# Autodesk Inventor assembly: 3dPrinter
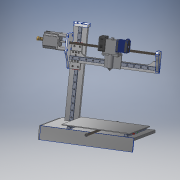
[picture p0: Inventor's stored thumbnail of the model, 180x180]
Saved by Autodesk Inventor 2019 (Build 230136000, 136)
## iProperties
Created: 2018-10-03
Part Number: 3dPrinter
Document SubType Name: Assembly
Designer: LillaHunden
Mass: 6608.48 g
Surface Area: 8581.85 cm^2
Volume: 2705.8 cm^3
Density: 2.44234 g/cm^3
Author: LillaHunden
## Documents named in this file (40)
- C:\Users\LillaHunden\Documents\Inventor\3dprinter\3dPrinter\3dPrinter.iam
- C:\Users\LillaHunden\Documents\Inventor\3dprinter\3dPrinter\baseplate.ipt
- C:\Users\LillaHunden\Documents\Inventor\3dprinter\3dPrinter\Zcolumn.ipt
- C:\Users\LillaHunden\Documents\Inventor\3dprinter\3dPrinter\ZcolStiffer.ipt
- C:\Users\LillaHunden\Documents\Inventor\3dprinter\3dPrinter\Linear Rials import\Rail Z.ipt
- C:\Users\LillaHunden\Documents\Inventor\3dprinter\3dPrinter\Linear Rials import\hotplate.ipt
- C:\Users\LillaHunden\Documents\Inventor\3dprinter\3dPrinter\Linear Rials import\MGN block.iam
- C:\Users\LillaHunden\Documents\Inventor\3dprinter\3dPrinter\Linear Rials import\Rail Y.ipt
- C:\Users\LillaHunden\Documents\Inventor\3dprinter\3dPrinter\Linear Rials import\Xcolum.ipt
- C:\Users\LillaHunden\Documents\Inventor\3dprinter\3dPrinter\Linear Rials import\XcolBracket.ipt
- C:\Users\LillaHunden\Documents\Inventor\3dprinter\3dPrinter\Linear Rials import\Rail X.ipt
- C:\Users\LillaHunden\Documents\Inventor\3dprinter\3dPrinter\Design Accelerator\Bolted Connection2.iam
- C:\Users\LillaHunden\Documents\Inventor\3dprinter\3dPrinter\Linear Rials import\Trapezoidal lead screw tr8x8-4 X.ipt
- C:\Users\LillaHunden\Documents\Inventor\3dprinter\3dPrinter\Linear Rials import\Trapezoidal lead screw tr8x8-4 Y.ipt
- C:\Users\LillaHunden\Documents\Inventor\3dprinter\3dPrinter\Linear Rials import\Trapezoidal lead screw tr8x8-4 Z.ipt
- C:\Users\LillaHunden\Documents\Inventor\3dprinter\3dPrinter\Linear Rials import\TR8_8(P4) Antibacklash Nut w. spring.ipt
- C:\Users\LillaHunden\Documents\Inventor\3dprinter\3dPrinter\Linear Rials import\ZnutBracket.ipt
- C:\Users\LillaHunden\Documents\Inventor\3dprinter\3dPrinter\Design Accelerator\Bolted Connection3.iam
- C:\Users\LillaHunden\Documents\Inventor\3dprinter\3dPrinter\Design Accelerator\Bolted Connection4.iam
- C:\Users\LillaHunden\Documents\Inventor\3dprinter\3dPrinter\ZBaringBracket.ipt
- C:\Users\LillaHunden\Documents\Inventor\3dprinter\3dPrinter\XMotorMount.ipt
- C:\Users\LillaHunden\Documents\Inventor\3dprinter\3dPrinter\23hs6403.ipt
- C:\Users\LillaHunden\Documents\Inventor\3dprinter\3dPrinter\Pulley import\GT2-20T-9mm\GT2_20T_9mm.ipt
- C:\Users\LillaHunden\Documents\Inventor\3dprinter\3dPrinter\XbearingBracket.ipt
- C:\Users\LillaHunden\Documents\Inventor\3dprinter\3dPrinter\3dPrinter\Design Accelerator\Bolted Connection1.iam
- C:\Users\LillaHunden\Documents\Inventor\3dprinter\3dPrinter\3dPrinter\Design Accelerator\Bolted Connection2.iam
- C:\Users\LillaHunden\Documents\Inventor\3dprinter\3dPrinter\3dPrinter\Design Accelerator\Bolted Connection3.iam
- C:\Users\LillaHunden\Documents\Inventor\3dprinter\3dPrinter\MR115 2RS.ipt
- C:\Users\LillaHunden\Documents\Inventor\3dprinter\3dPrinter\Extruder.iam
- C:\Users\LillaHunden\Documents\Inventor\3dprinter\3dPrinter\Extruder bracket.ipt
- C:\Users\LillaHunden\Documents\Inventor\Content Center Files\R2019\en-US\DIN 912\DIN 912 - M3 x 0,5 x 5 x 3,75.ipt
- C:\Users\LillaHunden\Documents\Inventor\3dprinter\3dPrinter\Frame Bottom Front.ipt
- C:\Users\LillaHunden\Documents\Inventor\3dprinter\3dPrinter\Frame bottom Left.ipt
- C:\Users\LillaHunden\Documents\Inventor\3dprinter\3dPrinter\3dPrinter\Design Accelerator\Bolted Connection4.iam
- C:\Users\LillaHunden\Documents\Inventor\3dprinter\3dPrinter\XMotorStandoff.ipt
- C:\Users\LillaHunden\Documents\Inventor\3dprinter\3dPrinter\3dPrinter\Design Accelerator\Bolted Connection6.iam
- C:\Users\LillaHunden\Documents\Inventor\3dprinter\3dPrinter\3dPrinter\Design Accelerator\Bolted Connection9.iam
- C:\Users\LillaHunden\Documents\Inventor\3dprinter\3dPrinter\3dPrinter\Design Accelerator\Bolted Connection10.iam
- C:\Users\LillaHunden\Documents\Inventor\3dprinter\3dPrinter\3dPrinter\Design Accelerator\Bolted Connection8.iam
- C:\Users\LillaHunden\Documents\Inventor\3dprinter\3dPrinter\XGuideBracket.ipt
## Components (63 placed, 29 different names)
1. baseplate:1 — Mate:20, Angle:1, Angle:2, Angle:3, Mate:32, Flush:16, Flush:17, Flush:25, Flush:26, Angle:11, Angle:12, Flush:40, Flush:41
2. Zcolumn:1 — Mate:11, Mate:12, Flush:8, Mate:20, Mate:21, Flush:9, Mate:22, Angle:3, Angle:4, Flush:25, Flush:26, Angle:7, Flush:30, Flush:31
3. ZcolStiffer:1 — Mate:11, Mate:12, Flush:8
4. Rail Z:1 — Mate:21, Flush:9, Mate:22, Mate:25, Mate:26, Mate:85, Mate:86
5. hotplate:1 — Mate:23, Mate:24, Flush:10, Flush:12, Angle:1, Angle:2, Flush:17, Angle:15
6. MGN block:1 [sub-assembly] — Mate:25, Angle:4, Mate:26, Flush:13, Mate:27, Flush:14, Flush:18, Flush:19, Flush:22, Mate:115, Mate:117
7. MGN block:2 [sub-assembly] — Flush:13, Mate:27, Flush:14
8. MGN block:3 [sub-assembly] — Mate:23, Flush:11, Symmetry:1, Flush:12, Mate:28, Mate:29
9. MGN block:4 [sub-assembly] — Mate:24, Flush:10, Flush:11, Symmetry:1, Mate:30, Mate:31
10. Rail Y:1 — Mate:30, Mate:31, Flush:15
11. Rail Y:2 — Mate:28, Mate:29, Flush:15, Mate:32, Flush:16, Angle:6
12. Xcolum:1 — Mate:33, Flush:20, Flush:21, Mate:34, Flush:23, Flush:24, Angle:5, Flush:29, Flush:36, Flush:37, Mate:116, Mate:118, Mate:119, Flush:44, Flush:45, Flush:49
13. XcolBracket:1 — Flush:18, Flush:19, Mate:33, Flush:20, Flush:21, Flush:22, Mate:50, Flush:33, Flush:34, Mate:114
14. Rail X:1 — Mate:34, Flush:23, Flush:24, Mate:35, Mate:36, Mate:102, Mate:103
15. MGN block:5 [sub-assembly] — Mate:35, Mate:36, Angle:16, Flush:39, Mate:76, Mate:77, Mate:125
16. Bolted Connection:1 [sub-assembly] — Mate:114, Mate:115
17. Trapezoidal lead screw tr8x8-4 X:1 — Angle:5, Mate:40, Mate:79, Mate:80
18. Trapezoidal lead screw tr8x8-4 Y:1 — Angle:6, Mate:41, Mate:58, Mate:73, Mate:74
19. Trapezoidal lead screw tr8x8-4 Z:1 — Angle:7, Mate:39, Mate:56, Mate:71
20. TR8_8(P4) Antibacklash Nut w. spring:1 — Mate:39, Mate:47, Mate:84
21. TR8_8(P4) Antibacklash Nut w. spring:2 — Mate:40
22. TR8_8(P4) Antibacklash Nut w. spring:3 — Mate:41
23. ZnutBracket:1 — Flush:29, Mate:47, Mate:83, Mate:104, Mate:105
24. Bolted Connection:2 [sub-assembly] — Mate:104, Mate:105
25. Bolted Connection:3 [sub-assembly] — Mate:83, Mate:84
26. ZBaringBracket:1 — Flush:30, Flush:31, Mate:61, Mate:62, Mate:63, Mate:64, Mate:69, Mate:70
27. XMotorMount:1 — Mate:50, Flush:33, Flush:34, Mate:78, Flush:42, Angle:17, Flush:43, Mate:120, Mate:121, Insert:9
28. 23hs6403:1 — Mate:78, Mate:79, Mate:80, Mate:93, Mate:94, Mate:95, Mate:96, Mate:97, Mate:98, Angle:17, Flush:43
29. 23hs6403:2 — Angle:12, Angle:13, Mate:57
30. 23hs6403:3 — Mate:56, Angle:11
31. GT2_20T_9mm:3 — Angle:14, Mate:58
32. GT2_20T_9mm:4 — Angle:13, Mate:57, Angle:14
33. XbearingBracket:1 — Flush:36, Flush:37, Flush:44, Flush:45, Mate:122, Mate:123, Mate:124
34. Bolted Connection:4 [sub-assembly] — Mate:61, Mate:62
35. Bolted Connection:5 [sub-assembly] — Mate:63, Mate:64
36. Bolted Connection:6 [sub-assembly] — Mate:85, Mate:86
37. MR115 2RS:1 — Mate:73
38. MR115 2RS:2 — Mate:122
39. MR115 2RS:3 — Mate:69, Mate:70, Mate:71
40. MR115 2RS:4 — Mate:74
41. Extruder:1 [sub-assembly] — Angle:15, Angle:16, Flush:38
42. Extruder bracket:1 — Flush:38, Insert:1, Insert:2, Insert:3, Insert:4, Insert:5, Insert:6, Insert:7, Insert:8, Flush:39, Mate:76, Mate:77, Flush:46, Flush:47, Flush:48
43. DIN 912 - replaced by DIN EN ISO 4762 M3 x 5:1 — Insert:1
44. DIN 912 - replaced by DIN EN ISO 4762 M3 x 5:2 — Insert:2
45. DIN 912 - replaced by DIN EN ISO 4762 M3 x 5:3 — Insert:3
46. DIN 912 - replaced by DIN EN ISO 4762 M3 x 5:4 — Insert:4
47. DIN 912 - replaced by DIN EN ISO 4762 M3 x 5:5 — Insert:5
48. DIN 912 - replaced by DIN EN ISO 4762 M3 x 5:6 — Insert:6
49. DIN 912 - replaced by DIN EN ISO 4762 M3 x 5:7 — Insert:7
50. DIN 912 - replaced by DIN EN ISO 4762 M3 x 5:8 — Insert:8
51. Frame Bottom Front:1 — Flush:40
52. Frame bottom Left:1 — Flush:41
53. Bolted Connection:7 [sub-assembly] — Mate:102, Mate:103
54. XMotorStandoff:1 — Flush:42
55. XMotorStandoff:2 — Mate:96, Mate:97
56. XMotorStandoff:3 — Mate:95, Mate:98
57. XMotorStandoff:4 — Mate:93, Mate:94
58. Bolted Connection:8 [sub-assembly] — Mate:120, Mate:121
59. Bolted Connection:10 [sub-assembly] — Mate:116, Mate:117
60. Bolted Connection:11 [sub-assembly] — Mate:118, Mate:119
61. MR115 2RS:5 — Insert:9
62. Bolted Connection:12 [sub-assembly] — Mate:123, Mate:124
63. XGuideBracket:1 — Mate:125, Flush:46, Flush:47, Flush:48, Flush:49
## Relationships (129: Mate 67, Flush 38, Angle 14, Insert 9, Symmetry 1)
- Mate:11: Zcolumn:1 ↔ ZcolStiffer:1
- Mate:12: Zcolumn:1 ↔ ZcolStiffer:1
- Flush:8: Zcolumn:1 ↔ ZcolStiffer:1
- Mate:20 (-5 mm): baseplate:1 ↔ Zcolumn:1
- Mate:21: Zcolumn:1 ↔ Rail Z:1
- Flush:9 (7 mm): Zcolumn:1 ↔ Rail Z:1
- Mate:22: Zcolumn:1 ↔ Rail Z:1
- Mate:23: hotplate:1 ↔ MGN block:3
- Mate:24: hotplate:1 ↔ MGN block:4
- Flush:10 (83 mm): hotplate:1 ↔ MGN block:4
- Flush:11: MGN block:3 ↔ MGN block:4
- Symmetry:1: MGN block:3 ↔ MGN block:4
- Flush:12 (7 mm): hotplate:1 ↔ MGN block:3
- Angle:1 (180 deg): baseplate:1 ↔ hotplate:1
- Angle:2 (90 deg): baseplate:1 ↔ hotplate:1
- Angle:3 (0 deg): baseplate:1 ↔ Zcolumn:1
- Mate:25: Rail Z:1 ↔ MGN block:1
- Angle:4 (0 deg): Zcolumn:1 ↔ MGN block:1
- Mate:26: Rail Z:1 ↔ MGN block:1
- Flush:13: MGN block:1 ↔ MGN block:2
- Mate:27 (7 mm): MGN block:1 ↔ MGN block:2
- Flush:14: MGN block:1 ↔ MGN block:2
- Mate:28: MGN block:3 ↔ Rail Y:2
- Mate:29: MGN block:3 ↔ Rail Y:2
- Mate:30: MGN block:4 ↔ Rail Y:1
- Mate:31: MGN block:4 ↔ Rail Y:1
- Flush:15: Rail Y:1 ↔ Rail Y:2
- Mate:32: baseplate:1 ↔ Rail Y:2
- Flush:16 (4 mm): baseplate:1 ↔ Rail Y:2
- Flush:17 (12 mm): baseplate:1 ↔ hotplate:1
- Flush:18: MGN block:1 ↔ XcolBracket:1
- Flush:19 (2.5 mm): MGN block:1 ↔ XcolBracket:1
- Mate:33: Xcolum:1 ↔ XcolBracket:1
- Flush:20: Xcolum:1 ↔ XcolBracket:1
- Flush:21 (25 mm): Xcolum:1 ↔ XcolBracket:1
- Flush:22 (-6.5 mm): MGN block:1 ↔ XcolBracket:1
- Mate:34: Xcolum:1 ↔ Rail X:1
- Flush:23: Xcolum:1 ↔ Rail X:1
- Flush:24 (10 mm): Xcolum:1 ↔ Rail X:1
- Mate:35: Rail X:1 ↔ MGN block:5
- Mate:36: Rail X:1 ↔ MGN block:5
- Flush:25 (26 mm): baseplate:1 ↔ Zcolumn:1
- Flush:26 (45 mm): baseplate:1 ↔ Zcolumn:1
- Angle:5 (0 deg): Xcolum:1 ↔ Trapezoidal lead screw tr8x8-4 X:1
- Angle:6 (0 deg): Rail Y:2 ↔ Trapezoidal lead screw tr8x8-4 Y:1
- Angle:7 (0 deg): Zcolumn:1 ↔ Trapezoidal lead screw tr8x8-4 Z:1
- Mate:39: Trapezoidal lead screw tr8x8-4 Z:1 ↔ TR8_8(P4) Antibacklash Nut w. spring:1
- Mate:40: Trapezoidal lead screw tr8x8-4 X:1 ↔ TR8_8(P4) Antibacklash Nut w. spring:2
- Mate:41: Trapezoidal lead screw tr8x8-4 Y:1 ↔ TR8_8(P4) Antibacklash Nut w. spring:3
- Flush:29: Xcolum:1 ↔ ZnutBracket:1
- Mate:47: TR8_8(P4) Antibacklash Nut w. spring:1 ↔ ZnutBracket:1
- Flush:30: Zcolumn:1 ↔ ZBaringBracket:1
- Flush:31: Zcolumn:1 ↔ ZBaringBracket:1
- Mate:50: XcolBracket:1 ↔ XMotorMount:1
- Flush:33: XcolBracket:1 ↔ XMotorMount:1
- Flush:34 (10 mm): XcolBracket:1 ↔ XMotorMount:1
- Mate:56: Trapezoidal lead screw tr8x8-4 Z:1 ↔ 23hs6403:3
- Angle:11 (0 deg): baseplate:1 ↔ 23hs6403:3
- Angle:12 (0 deg): baseplate:1 ↔ 23hs6403:2
- Angle:13 (0 deg): 23hs6403:2 ↔ GT2_20T_9mm:4
- Mate:57: 23hs6403:2 ↔ GT2_20T_9mm:4
- Angle:14 (0 deg): GT2_20T_9mm:3 ↔ GT2_20T_9mm:4
- Mate:58: Trapezoidal lead screw tr8x8-4 Y:1 ↔ GT2_20T_9mm:3
- Flush:36: Xcolum:1 ↔ XbearingBracket:1
- Flush:37: Xcolum:1 ↔ XbearingBracket:1
- Mate:61: ZBaringBracket:1 ↔ Bolted Connection:4
- Mate:62: ZBaringBracket:1 ↔ Bolted Connection:4
- Mate:63: ZBaringBracket:1 ↔ Bolted Connection:5
- Mate:64: ZBaringBracket:1 ↔ Bolted Connection:5
- Mate:69: ZBaringBracket:1 ↔ MR115 2RS:3
- Mate:70: ZBaringBracket:1 ↔ MR115 2RS:3
- Mate:71: Trapezoidal lead screw tr8x8-4 Z:1 ↔ MR115 2RS:3
- Mate:73: Trapezoidal lead screw tr8x8-4 Y:1 ↔ MR115 2RS:1
- Mate:74: Trapezoidal lead screw tr8x8-4 Y:1 ↔ MR115 2RS:4
- Angle:15 (180 deg): hotplate:1 ↔ Extruder:1
- Angle:16 (180 deg): MGN block:5 ↔ Extruder:1
- Flush:38: Extruder:1 ↔ Extruder bracket:1
- Insert:1: Extruder bracket:1 ↔ DIN 912 - replaced by DIN EN ISO 4762 M3 x 5:1
- Insert:2: Extruder bracket:1 ↔ DIN 912 - replaced by DIN EN ISO 4762 M3 x 5:2
- Insert:3: Extruder bracket:1 ↔ DIN 912 - replaced by DIN EN ISO 4762 M3 x 5:3
- Insert:4: Extruder bracket:1 ↔ DIN 912 - replaced by DIN EN ISO 4762 M3 x 5:4
- Insert:5: Extruder bracket:1 ↔ DIN 912 - replaced by DIN EN ISO 4762 M3 x 5:5
- Insert:6: Extruder bracket:1 ↔ DIN 912 - replaced by DIN EN ISO 4762 M3 x 5:6
- Insert:7: Extruder bracket:1 ↔ DIN 912 - replaced by DIN EN ISO 4762 M3 x 5:7
- Insert:8: Extruder bracket:1 ↔ DIN 912 - replaced by DIN EN ISO 4762 M3 x 5:8
- Flush:39 (5 mm): MGN block:5 ↔ Extruder bracket:1
- Mate:76 (20 mm): MGN block:5 ↔ Extruder bracket:1
- Mate:77 (5 mm): MGN block:5 ↔ Extruder bracket:1
- Flush:40: baseplate:1 ↔ Frame Bottom Front:1
- Flush:41: baseplate:1 ↔ Frame bottom Left:1
- Mate:78 (30 mm): XMotorMount:1 ↔ 23hs6403:1
- Mate:79: Trapezoidal lead screw tr8x8-4 X:1 ↔ 23hs6403:1
- Mate:80 (5 mm): Trapezoidal lead screw tr8x8-4 X:1 ↔ 23hs6403:1
- Mate:83: ZnutBracket:1 ↔ Bolted Connection:3
- Mate:84: TR8_8(P4) Antibacklash Nut w. spring:1 ↔ Bolted Connection:3
- Mate:85: Rail Z:1 ↔ Bolted Connection:6
- Mate:86: Rail Z:1 ↔ Bolted Connection:6
- Flush:42: XMotorMount:1 ↔ XMotorStandoff:1
- Mate:93: 23hs6403:1 ↔ XMotorStandoff:4
- Mate:94: 23hs6403:1 ↔ XMotorStandoff:4
- Mate:95: 23hs6403:1 ↔ XMotorStandoff:3
- Mate:96: 23hs6403:1 ↔ XMotorStandoff:2
- Mate:97: 23hs6403:1 ↔ XMotorStandoff:2
- Mate:98: 23hs6403:1 ↔ XMotorStandoff:3
- Angle:17 (0 deg): XMotorMount:1 ↔ 23hs6403:1
- Mate:102: Rail X:1 ↔ Bolted Connection:7
- Mate:103: Rail X:1 ↔ Bolted Connection:7
- Flush:43 (5.2 mm): XMotorMount:1 ↔ 23hs6403:1
- Mate:104: ZnutBracket:1 ↔ Bolted Connection:2
- Mate:105: ZnutBracket:1 ↔ Bolted Connection:2
- Mate:114: XcolBracket:1 ↔ Bolted Connection:1
- Mate:115: MGN block:1 ↔ Bolted Connection:1
- Mate:116: Xcolum:1 ↔ Bolted Connection:10
- Mate:117: MGN block:1 ↔ Bolted Connection:10
- Mate:118: Xcolum:1 ↔ Bolted Connection:11
- Mate:119: Xcolum:1 ↔ Bolted Connection:11
- Mate:120: XMotorMount:1 ↔ Bolted Connection:8
- Mate:121: XMotorMount:1 ↔ Bolted Connection:8
- Insert:9: XMotorMount:1 ↔ MR115 2RS:5
- Flush:44: Xcolum:1 ↔ XbearingBracket:1
- Flush:45: Xcolum:1 ↔ XbearingBracket:1
- Mate:122: XbearingBracket:1 ↔ MR115 2RS:2
- Mate:123: XbearingBracket:1 ↔ Bolted Connection:12
- Mate:124: XbearingBracket:1 ↔ Bolted Connection:12
- Mate:125: MGN block:5 ↔ XGuideBracket:1
- Flush:46: Extruder bracket:1 ↔ XGuideBracket:1
- Flush:47: Extruder bracket:1 ↔ XGuideBracket:1
- Flush:48: Extruder bracket:1 ↔ XGuideBracket:1
- Flush:49: Xcolum:1 ↔ XGuideBracket:1
